# Autodesk Inventor assembly: bloczki
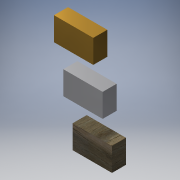
[picture p0: Inventor's stored thumbnail of the model, 180x180]
Saved by Autodesk Inventor 2018.3 (Build 223284000, 284)
## iProperties
Created: 2020-04-19
Part Number: bloczki
Material: Ogólny
Document SubType Name: Assembly
Designer: Wojciech
Author: Wojciech
## Documents named in this file (2)
- C:\Users\Wojciech\OneDrive\Documents\studia\labki 2020\101\bloczki.iam
- C:\Users\Wojciech\OneDrive\Documents\studia\labki 2020\101\kloc.ipt
## Components (3 placed, 1 different names)
1. kloc:1 — Równoległy:1, Równoległy:2, Równoległy:3, Równoległy:4, Zestawiający:2, Zestawiający:3
2. kloc:2 — Równoległy:1, Równoległy:4, Zestawiający:3
3. kloc:3 — Równoległy:2, Zestawiający:1, Równoległy:3, Zestawiający:2
## Relationships (7: Flush 4, Mate 3)
- Równoległy:1 [Flush]: kloc:1 ↔ kloc:2
- Równoległy:2 [Flush]: kloc:1 ↔ kloc:3
- Zestawiający:1 [Mate]: kloc:3
- Równoległy:3 [Flush] (10 mm): kloc:1 ↔ kloc:3
- Równoległy:4 [Flush] (10 mm): kloc:1 ↔ kloc:2
- Zestawiający:2 [Mate] (20 mm): kloc:1 ↔ kloc:3
- Zestawiający:3 [Mate] (20 mm): kloc:1 ↔ kloc:2
